# Autodesk Inventor assembly: Arm_Left
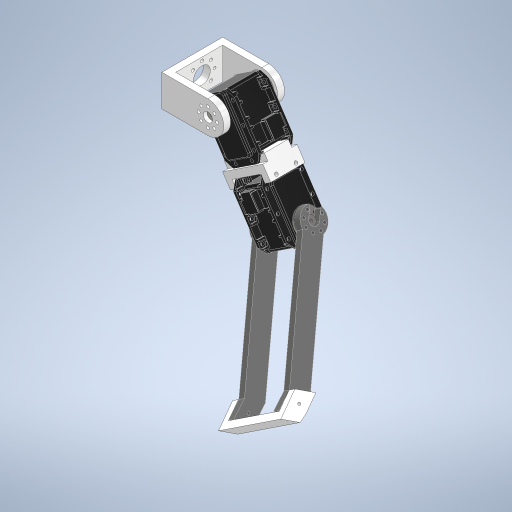
[picture p0: Inventor's stored thumbnail of the model, 512x512]
Saved by Autodesk Inventor 2024.3 (Build 283343000, 343)
## iProperties
Created: 2024-09-18
Part Number: Arm_Left
Document SubType Name: Assembly
Designer: 구지현
Author: 구지현
## Documents named in this file (8)
- C:\Users\구지현\Desktop\19th_intern_kdy_robot\부품\Upper_Body\Arm\Arm_Left.iam
- C:\Users\구지현\Desktop\19th_intern_kdy_robot\부품\Upper_Body\Arm\Hand_Connection_Parts.ipt
- C:\Users\구지현\Desktop\19th_intern_kdy_robot\부품\Upper_Body\Arm\Middle_Arm_Fixing_Parts.ipt
- C:\Users\구지현\Desktop\19th_intern_kdy_robot\부품\Upper_Body\Arm\Shoulder_Fixing_Parts_Left.ipt
- C:\Users\구지현\Desktop\19th_intern_kdy_robot\부품\Upper_Body\Arm\Hand.ipt
- C:\Users\구지현\Documents\카카오톡 받은 파일\Hardware\ROBOTIS(Inventor 2024 ver.)\다이나믹셀\MX-28T_R+idle.ipt.iam
- C:\Users\구지현\Documents\카카오톡 받은 파일\Hardware\ROBOTIS(Inventor 2024 ver.)\혼\28Horn.ipt
- MX-28T_R+idle.ipt
## Components (8 placed, 6 different names)
1. Hand:1 — 메이트:1, 메이트:2, 삽입:10
2. Hand_Connection_Parts:1 — 삽입:10
3. Middle_Arm_Fixing_Parts:1 — 삽입:4, 삽입:5, 삽입:6, 삽입:7, 삽입:8, 삽입:9
4. Shoulder_Fixing_Parts_Left:1 — 삽입:3
5. MX-28T_R+idle.ipt:3 [sub-assembly] — 삽입:2, 삽입:4, 삽입:5
6. MX-28T_R+idle.ipt:4 [sub-assembly] — 삽입:1, 삽입:6, 삽입:7, 삽입:8, 삽입:9
7. 28Horn:1 — 삽입:2, 삽입:3
8. 28Horn:2 — 삽입:1, 메이트:1, 메이트:2
## Relationships (12: Insert 10, Mate 2)
- 삽입:1 [Insert]: MX-28T_R+idle.ipt:4 ↔ 28Horn:2
- 삽입:2 [Insert]: MX-28T_R+idle.ipt:3 ↔ 28Horn:1
- 삽입:3 [Insert]: Shoulder_Fixing_Parts_Left:1 ↔ 28Horn:1
- 삽입:4 [Insert]: Middle_Arm_Fixing_Parts:1 ↔ MX-28T_R+idle.ipt:3
- 삽입:5 [Insert]: Middle_Arm_Fixing_Parts:1 ↔ MX-28T_R+idle.ipt:3
- 삽입:6 [Insert]: Middle_Arm_Fixing_Parts:1 ↔ MX-28T_R+idle.ipt:4
- 삽입:7 [Insert]: Middle_Arm_Fixing_Parts:1 ↔ MX-28T_R+idle.ipt:4
- 삽입:8 [Insert]: Middle_Arm_Fixing_Parts:1 ↔ MX-28T_R+idle.ipt:4
- 삽입:9 [Insert]: Middle_Arm_Fixing_Parts:1 ↔ MX-28T_R+idle.ipt:4
- 메이트:1 [Mate]: Hand:1 ↔ 28Horn:2
- 메이트:2 [Mate]: Hand:1 ↔ 28Horn:2
- 삽입:10 [Insert]: Hand:1 ↔ Hand_Connection_Parts:1
